# Autodesk Inventor assembly: pcb stack
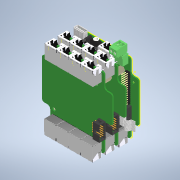
[picture p0: Inventor's stored thumbnail of the model, 180x180]
Saved by Autodesk Inventor 2021 (Build 250183000, 183)
## iProperties
Created: 2023-08-07
Part Number: pcb stack
Document SubType Name: Assembly
Designer: michal
Author: michal
## Documents named in this file (4)
- C:\Users\micha\OneDrive\Dokumenty\GitHub\escape_room_hw_v2\Enclosure\Commercial\pcb stack.iam
- C:\Users\micha\OneDrive\Dokumenty\GitHub\escape_room_hw_v2\Enclosure\Commercial\dystans 20mm.ipt
- C:\Users\micha\OneDrive\Dokumenty\GitHub\escape_room_hw_v2\Enclosure\pcbwitchElements.iam
- C:\Users\micha\OneDrive\Dokumenty\GitHub\escape_room_hw_v2\Enclosure\pcbIOExt.iam
## Components (11 placed, 3 different names)
1. dystans 20mm:1 — Mate:1, Mate:8, Mate:28
2. pcbwitchElements:1 [sub-assembly] — Mate:1, Mate:2, Mate:3, Mate:4, Mate:5, Mate:6, Mate:7, Mate:8
3. dystans 20mm:2 — Mate:2, Mate:7, Mate:11, Mate:27
4. dystans 20mm:3 — Mate:3, Mate:6, Mate:12, Mate:25
5. dystans 20mm:4 — Mate:4, Mate:5, Mate:13, Mate:26
6. pcbIOExt:1 [sub-assembly] — Mate:11, Mate:12, Mate:13, Mate:29, Mate:30, Mate:31
7. dystans 20mm:5 — Mate:28, Mate:31
8. dystans 20mm:6 — Mate:27, Mate:30
9. dystans 20mm:7 — Mate:25, Mate:32
10. dystans 20mm:8 — Mate:26, Mate:29
11. pcbIOExt:2 [sub-assembly] — Mate:32
## Relationships (22: Mate 22)
- Mate:1: dystans 20mm:1 ↔ pcbwitchElements:1
- Mate:2: pcbwitchElements:1 ↔ dystans 20mm:2
- Mate:3: pcbwitchElements:1 ↔ dystans 20mm:3
- Mate:4: pcbwitchElements:1 ↔ dystans 20mm:4
- Mate:5: pcbwitchElements:1 ↔ dystans 20mm:4
- Mate:6: pcbwitchElements:1 ↔ dystans 20mm:3
- Mate:7: pcbwitchElements:1 ↔ dystans 20mm:2
- Mate:8: dystans 20mm:1 ↔ pcbwitchElements:1
- Mate:11: dystans 20mm:2 ↔ pcbIOExt:1
- Mate:12: dystans 20mm:3 ↔ pcbIOExt:1
- Mate:13: dystans 20mm:4 ↔ pcbIOExt:1
- [Mate]: dystans 20mm:6 ↔ pcbIOExt:2
- [Mate]: dystans 20mm:7 ↔ pcbIOExt:2
- [Mate]: dystans 20mm:8 ↔ pcbIOExt:2
- Mate:25: dystans 20mm:3 ↔ dystans 20mm:7
- Mate:26: dystans 20mm:4 ↔ dystans 20mm:8
- Mate:27: dystans 20mm:2 ↔ dystans 20mm:6
- Mate:28: dystans 20mm:1 ↔ dystans 20mm:5
- Mate:29: pcbIOExt:1 ↔ dystans 20mm:8
- Mate:30: pcbIOExt:1 ↔ dystans 20mm:6
- Mate:31: pcbIOExt:1 ↔ dystans 20mm:5
- Mate:32: dystans 20mm:7 ↔ pcbIOExt:2
## Named parameters: d15_d13 = 0 mm, d16_d14 = 0 mm, d25_d12 = 0 mm
